# Autodesk Inventor assembly: armsteun rechts
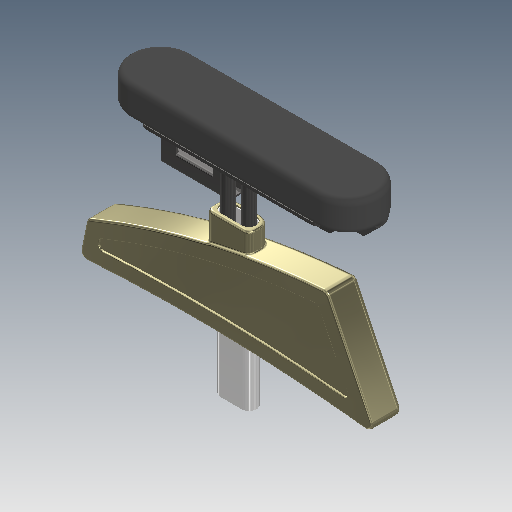
[picture p0: Inventor's stored thumbnail of the model, 512x512]
Saved by Autodesk Inventor 2020.3 (Build 243373000, 373)
## iProperties
Created: 2020-09-11
Part Number: armsteun rechts
Document SubType Name: Assembly
Designer: Svend
Author: Svend
## Documents named in this file (6)
- C:\Users\Svend\OneDrive\Documents\GitHub\Rolstoel\armsteun rechts.iam
- C:\Users\Svend\OneDrive\Documents\GitHub\Rolstoel\armsteun houder rechts.ipt
- C:\Users\Svend\OneDrive\Documents\GitHub\Rolstoel\armsteun.ipt
- C:\Users\Svend\OneDrive\Documents\GitHub\Rolstoel\beugel armsteun.ipt
- C:\Users\Svend\OneDrive\Documents\GitHub\Rolstoel\buis armsteun.ipt
- C:\Users\Svend\OneDrive\Documents\GitHub\Rolstoel\profiel armsteun.ipt
## Components (5 placed, 5 different names)
1. armsteun houder rechts:1 — Mate:7, Mate:8, Mate:9, Angle:1, Mate:11
2. armsteun:1 — Mate:1, Mate:2, Mate:3, Angle:1
3. beugel armsteun:1 — Mate:1, Mate:2, Mate:3, Mate:4, Mate:5, Mate:6, Mate:10, Mate:11
4. buis armsteun:1 — Mate:7, Mate:8, Mate:9, Mate:10
5. profiel armsteun:1 — Mate:4, Mate:5, Mate:6
## Relationships (12: Mate 11, Angle 1)
- Mate:1: armsteun:1 ↔ beugel armsteun:1
- Mate:2: armsteun:1 ↔ beugel armsteun:1
- Mate:3: armsteun:1 ↔ beugel armsteun:1
- Mate:4: beugel armsteun:1 ↔ profiel armsteun:1
- Mate:5: beugel armsteun:1 ↔ profiel armsteun:1
- Mate:6: beugel armsteun:1 ↔ profiel armsteun:1
- Mate:7: armsteun houder rechts:1 ↔ buis armsteun:1
- Mate:8: armsteun houder rechts:1 ↔ buis armsteun:1
- Mate:9 (2 mm): armsteun houder rechts:1 ↔ buis armsteun:1
- Mate:10: beugel armsteun:1 ↔ buis armsteun:1
- Angle:1 (0 deg): armsteun houder rechts:1 ↔ armsteun:1
- Mate:11 (50 mm): armsteun houder rechts:1 ↔ beugel armsteun:1
